# Autodesk Inventor assembly: Tanque5G
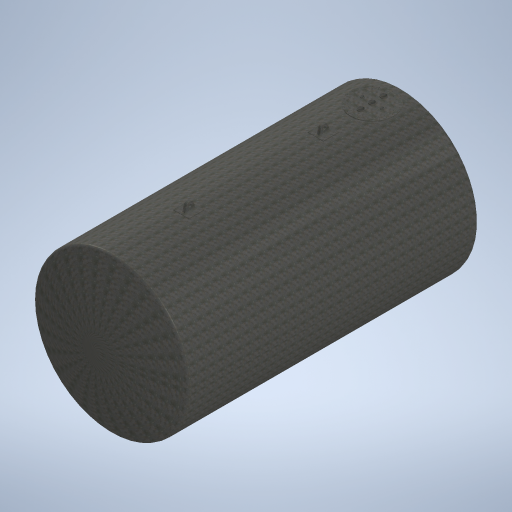
[picture p0: Inventor's stored thumbnail of the model, 512x512]
Saved by Autodesk Inventor 2023 (Build 270158000, 158)
## iProperties
Created: 2022-11-02
Part Number: Tanque5G
Document SubType Name: Assembly
Designer: Juanse
Author: Juanse
## Documents named in this file (5)
- C:\Users\Personal\Downloads\Modelado_Tanque\Workspaces\Workspace\Tanque5G.iam
- C:\Users\Personal\Downloads\Modelado_Tanque\Workspaces\Workspace\Tanque5000.ipt
- C:\Users\Personal\Downloads\Modelado_Tanque\Workspaces\Workspace\Brida_cuello_tapa.ipt
- C:\Users\Personal\Downloads\Modelado_Tanque\Workspaces\Workspace\Tapa1.ipt
- C:\Users\Personal\Downloads\Modelado_Tanque\Workspaces\Workspace\Tapa2.ipt
## Components (4 placed, 4 different names)
1. Tanque5000:1 — Mate:1, Flush:3, Mate:3, Mate:4, Mate:6
2. Brida_cuello_tapa:1 — Mate:4, Mate:5, Mate:6, Mate:7, Mate:8, Mate:9, Mate:10, Mate:11, Mate:12
3. Tapa1:1 — Mate:7, Mate:8, Mate:9
4. Tapa2:1 — Mate:10, Mate:11, Mate:12
## Relationships (12: Mate 11, Flush 1)
- Mate:1: Tanque5000:1
- Flush:3: Tanque5000:1
- Mate:3: Tanque5000:1
- Mate:4: Tanque5000:1 ↔ Brida_cuello_tapa:1
- Mate:5: Brida_cuello_tapa:1
- Mate:6: Tanque5000:1 ↔ Brida_cuello_tapa:1
- Mate:7: Brida_cuello_tapa:1 ↔ Tapa1:1
- Mate:8: Brida_cuello_tapa:1 ↔ Tapa1:1
- Mate:9: Brida_cuello_tapa:1 ↔ Tapa1:1
- Mate:10: Brida_cuello_tapa:1 ↔ Tapa2:1
- Mate:11: Brida_cuello_tapa:1 ↔ Tapa2:1
- Mate:12: Brida_cuello_tapa:1 ↔ Tapa2:1
